# Autodesk Inventor assembly: majk
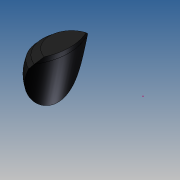
[picture p0: Inventor's stored thumbnail of the model, 180x180]
Saved by Autodesk Inventor 2012 (Build 160160000, 160)
## iProperties
Created: 2011-12-04
Part Number: majk
Document SubType Name: Assembly
Designer: slazh bliskovic
Author: slazh bliskovic
## Documents named in this file (3)
- C:\Users\BOZIDAR\Documents\Inventor\quickcam pro 9000\majk.iam
- C:\Users\BOZIDAR\Documents\Inventor\quickcam pro 9000\gornji shiny dio - Copy.ipt
- C:\Users\BOZIDAR\Documents\Inventor\quickcam pro 9000\kamerica - Copy.ipt
## Components (2 placed, 2 different names)
1. gornji shiny dio - Copy:1 — Mate:1, Mate:2
2. kamerica - Copy:1 — Mate:1, Mate:2
## Relationships (2: Mate 2)
- Mate:1: gornji shiny dio - Copy:1 ↔ kamerica - Copy:1
- Mate:2: gornji shiny dio - Copy:1 ↔ kamerica - Copy:1
